# Autodesk Inventor assembly: 276-2154
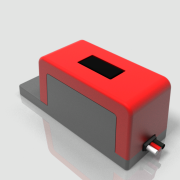
[picture p0: Inventor's stored thumbnail of the model, 180x180]
Saved by Autodesk Inventor 2013 (Build 170138000, 138)
## iProperties
Category: Sensors
Company: Super Sonic Sparks, Team 24
Part Number: 276-2154
Document SubType Name: Assembly
Designer: Jordan Kiesel
Mass: 15.422 g
Surface Area: 90.1 cm^2
Volume: 6.59444 cm^3
Catalog Web Link: vexrobotics.com/276-2154.html
Description: Program your robot to follow a black line over a white surface.
Vendor: VEX Robotics, Inc.
Translation Standard: STEP AP203
FileName: Line Tracker.iam
PreProcessor: SolidWorks 2006052
PostProcessor: Build: 239, Release: 2011 RTM - Date: Wed 02/17/2010
Sent Units: inch
Uncertainty: 1e-05
Author: Jordan Kiesel
Title: Line Tracker
Comments: Program your robot to follow a black line over a white surface. This kit provides more design flexibility--you can also use it to program your robot for light sensing. A Programming Kit is needed to change the program in the VEX Controller. ▷ Navigate down a marked path. ▷ Use for light sensing. ▷ More autonomous function.
## Documents named in this file (6)
- C:\Users\WEBCAST2\Documents\New VEX CAD Parts\Motors & Sensors\Line Tracker (Old).iam
- C:\Users\WEBCAST2\Documents\New VEX CAD Parts\Motors & Sensors\Assembly Parts\Line Tracker (Old)\Bottom.ipt
- C:\Users\WEBCAST2\Documents\New VEX CAD Parts\Motors & Sensors\Assembly Parts\Line Tracker (Old)\Sensor.ipt
- C:\Users\WEBCAST2\Documents\New VEX CAD Parts\Motors & Sensors\Assembly Parts\Line Tracker (Old)\Top.ipt
- C:\Users\WEBCAST2\Documents\New VEX CAD Parts\Motors & Sensors\Assembly Parts\Sensors\Wire Sleeve.ipt
- C:\Users\WEBCAST2\Documents\New VEX CAD Parts\Motors & Sensors\Assembly Parts\Sensors\3-Wire Black-Red-White Cable-Cut.ipt
## Components (5 placed, 5 different names)
1. Bottom:1 — Mate:1, Mate:2, Mate:3
2. Sensor:1
3. Top:1 — Mate:1, Mate:2, Mate:3
4. Wire Sleeve:1 — Angle:1, Tangent:1, Tangent:2, Tangent:3
5. 3-Wire Black-Red-White Cable-Cut:1 — Angle:1, Tangent:1, Tangent:2, Tangent:3
## Relationships (7: Mate 3, Tangent 3, Angle 1)
- Mate:1: Bottom:1 ↔ Top:1
- Mate:2: Bottom:1 ↔ Top:1
- Mate:3: Bottom:1 ↔ Top:1
- Angle:1 (0 deg): Wire Sleeve:1 ↔ 3-Wire Black-Red-White Cable-Cut:1
- Tangent:1 (0.1143 mm): Wire Sleeve:1 ↔ 3-Wire Black-Red-White Cable-Cut:1
- Tangent:2 (0.1143 mm): Wire Sleeve:1 ↔ 3-Wire Black-Red-White Cable-Cut:1
- Tangent:3 (0.2159 mm): Wire Sleeve:1 ↔ 3-Wire Black-Red-White Cable-Cut:1
